# Autodesk Inventor assembly: 2AM-17-A-5200 - claw
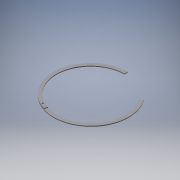
[picture p0: Inventor's stored thumbnail of the model, 180x180]
Saved by Autodesk Inventor 2017 (Build 210142000, 142)
## iProperties
Created: 2017-12-27
Part Number: 2AM-17-A-5200 - claw
Document SubType Name: Assembly
Designer: Micah
Author: Micah
## Documents named in this file (3)
- C:\Users\Micah\Desktop\inventor\CADathon-2017\2AM-17-A-0200 - Smokestack Elevator\2AM-17-A-5200 - claw.iam
- C:\Users\Micah\Desktop\inventor\CADathon-2017\2AM-17-A-0200 - Smokestack Elevator\2AM-17-P-5201 - claw part.ipt
- C:\Users\Micah\Desktop\inventor\CADathon-2017\2AM-17-A-0200 - Smokestack Elevator\2AM-17-P-5202 - claw part right.ipt
## Components (2 placed, 2 different names)
1. 2AM-17-P-5201 - claw part:1 — Rotational:1
2. 2AM-17-P-5202 - claw part right:1 — Rotational:1
## Relationships (1: RevoluteJoint 1)
- Rotational:1 [RevoluteJoint]: 2AM-17-P-5201 - claw part:1 ↔ 2AM-17-P-5202 - claw part right:1
